# Autodesk Inventor assembly: carriage
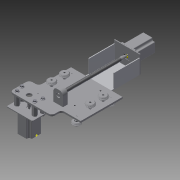
[picture p0: Inventor's stored thumbnail of the model, 180x180]
Saved by Autodesk Inventor 2013 (Build 170138000, 138)
## iProperties
Created: 2012-12-03
Part Number: carriage
Document SubType Name: Weldment
Designer: Istvan
Weld Material: Aluminum 6061, Welded
Mass: 772.809 g
Surface Area: 2087.48 cm^2
Volume: 764.052 cm^3
Density: 1.01146 g/cm^3
Author: Istvan
## Documents named in this file (14)
- C:\Users\james.eddlestone\Documents\GitHub\Crown-Fire\CAD\Carriage\carriage.iam
- C:\Users\james.eddlestone\Documents\GitHub\Crown-Fire\CAD\Carriage\backplate.ipt
- C:\Users\james.eddlestone\Documents\GitHub\Crown-Fire\CAD\Hardware\Bearings\DualVee-size2.ipt
- C:\Users\james.eddlestone\Documents\GitHub\Crown-Fire\CAD\Electronics\Motors\G723-280-4.ipt
- C:\Users\james.eddlestone\Documents\GitHub\Crown-Fire\CAD\Carriage\zMotorMount.ipt
- C:\Users\james.eddlestone\Documents\GitHub\Crown-Fire\CAD\Carriage\acmeScrew.ipt
- C:\Users\james.eddlestone\Documents\GitHub\Crown-Fire\CAD\Hardware\motorCoupling.ipt
- C:\Users\james.eddlestone\Documents\GitHub\Crown-Fire\CAD\Carriage\acmeBearingBlock.ipt
- C:\Users\james.eddlestone\Documents\GitHub\Crown-Fire\CAD\Carriage\motorMount.ipt
- C:\Users\james.eddlestone\Documents\GitHub\Crown-Fire\CAD\Hardware\1-4-20Standoff.ipt
- C:\Users\james.eddlestone\Documents\GitHub\Crown-Fire\CAD\Hardware\Fasteners\IFI 111 - 1_4-20 UNC x 0.5.ipt
- C:\Users\james.eddlestone\Documents\GitHub\Crown-Fire\CAD\Hardware\Bearings\10mm-double.ipt
- C:\Users\james.eddlestone\Documents\GitHub\Crown-Fire\CAD\CuttingHead\motorTower.ipt
- C:\Users\istvan.burbank\Documents\GitHub\Crown-Fire\CAD\Templates\channel2.25x4.ipt
## Components (31 placed, 12 different names)
1. backplate:1 — Mate:18, Mate:19, Mate:20, Mate:21, Mate:22, Mate:23, Mate:24, Mate:25, Mate:32, Mate:33, Mate:34, Mate:35, Mate:36, Insert:35, Mate:46, Insert:36, Insert:37, Insert:38, Insert:39, Mate:49, Flush:7, Mate:50, Flush:10
2. DualVee-size2:1 — Mate:18
3. DualVee-size2:2 — Mate:19
4. DualVee-size2:3 — Mate:21
5. DualVee-size2:4 — Mate:20
6. G723-280-4:1 — Mate:6, Mate:7, Mate:8, Mate:10, Flush:6, Angle:3
7. zMotorMount:1 — Mate:6, Mate:7, Angle:3, Mate:51, Flush:8, Flush:9
8. acmeScrew:1 — Mate:9, Mate:10, Flush:6, Mate:12, Mate:40, Mate:41, Mate:44
9. motorCoupling:1 — Mate:8, Mate:9, Mate:44
10. acmeBearingBlock:1 — Mate:12, Mate:39, Mate:49, Flush:7
11. DualVee-size2:5 — Mate:24
12. DualVee-size2:6 — Mate:23
13. DualVee-size2:7 — Mate:25
14. DualVee-size2:8 — Mate:22
15. G723-280-4:2 — Mate:31, Mate:32, Insert:32, Mate:45, Angle:2
16. motorMount:1 — Insert:19, Insert:20, Insert:28, Insert:29, Insert:30, Insert:31, Mate:45, Insert:33, Insert:34, Angle:2
17. motorCoupling:2 — Mate:31, Insert:32
18. 1-4-20Standoff:1 — Mate:35, Insert:34
19. 1-4-20Standoff:2 — Mate:33, Insert:33
20. 1-4-20Standoff:3 — Mate:36, Insert:29, Mate:46
21. 1-4-20Standoff:4 — Mate:34, Insert:28, Insert:35
22. Hex Flange Screw - Inch (IFI) 1/4-20 UNC x 0.5:1 — Insert:20
23. Hex Flange Screw - Inch (IFI) 1/4-20 UNC x 0.5:2 — Insert:19
24. Hex Flange Screw - Inch (IFI) 1/4-20 UNC x 0.5:3 — Insert:30
25. Hex Flange Screw - Inch (IFI) 1/4-20 UNC x 0.5:4 — Insert:31
26. Hex Flange Screw - Inch (IFI) 1/4-20 UNC x 0.5:5 — Insert:39
27. Hex Flange Screw - Inch (IFI) 1/4-20 UNC x 0.5:6 — Insert:37
28. Hex Flange Screw - Inch (IFI) 1/4-20 UNC x 0.5:7 — Insert:38
29. Hex Flange Screw - Inch (IFI) 1/4-20 UNC x 0.5:8 — Insert:36
30. 10mm-double:1 — Mate:39, Mate:40, Mate:41
31. motorTower:1 — Mate:50, Mate:51, Flush:8, Flush:9, Flush:10
## Relationships (50: Mate 29, Insert 14, Flush 5, Angle 2)
- Mate:6: G723-280-4:1 ↔ zMotorMount:1
- Mate:7: G723-280-4:1 ↔ zMotorMount:1
- Mate:8: G723-280-4:1 ↔ motorCoupling:1
- Mate:9: acmeScrew:1 ↔ motorCoupling:1
- Mate:10: G723-280-4:1 ↔ acmeScrew:1
- Flush:6: G723-280-4:1 ↔ acmeScrew:1
- Mate:12: acmeScrew:1 ↔ acmeBearingBlock:1
- Mate:18: backplate:1 ↔ DualVee-size2:1
- Mate:19: backplate:1 ↔ DualVee-size2:2
- Mate:20: backplate:1 ↔ DualVee-size2:4
- Mate:21: backplate:1 ↔ DualVee-size2:3
- Mate:22: backplate:1 ↔ DualVee-size2:8
- Mate:23: backplate:1 ↔ DualVee-size2:6
- Mate:24: backplate:1 ↔ DualVee-size2:5
- Mate:25: backplate:1 ↔ DualVee-size2:7
- Mate:31: G723-280-4:2 ↔ motorCoupling:2
- Mate:32: backplate:1 ↔ G723-280-4:2
- Mate:33: backplate:1 ↔ 1-4-20Standoff:2
- Mate:34: backplate:1 ↔ 1-4-20Standoff:4
- Mate:35: backplate:1 ↔ 1-4-20Standoff:1
- Mate:36: backplate:1 ↔ 1-4-20Standoff:3
- Insert:19: motorMount:1 ↔ Hex Flange Screw - Inch (IFI) 1/4-20 UNC x 0.5:2
- Insert:20: motorMount:1 ↔ Hex Flange Screw - Inch (IFI) 1/4-20 UNC x 0.5:1
- Insert:28: motorMount:1 ↔ 1-4-20Standoff:4
- Insert:29: motorMount:1 ↔ 1-4-20Standoff:3
- Insert:30: motorMount:1 ↔ Hex Flange Screw - Inch (IFI) 1/4-20 UNC x 0.5:3
- Insert:31: motorMount:1 ↔ Hex Flange Screw - Inch (IFI) 1/4-20 UNC x 0.5:4
- Insert:32 (-12.7 mm): G723-280-4:2 ↔ motorCoupling:2
- Mate:39: acmeBearingBlock:1 ↔ 10mm-double:1
- Mate:40: acmeScrew:1 ↔ 10mm-double:1
- Mate:41: acmeScrew:1 ↔ 10mm-double:1
- Mate:44: acmeScrew:1 ↔ motorCoupling:1
- Mate:45: G723-280-4:2 ↔ motorMount:1
- Insert:33: motorMount:1 ↔ 1-4-20Standoff:2
- Insert:34: motorMount:1 ↔ 1-4-20Standoff:1
- Insert:35: backplate:1 ↔ 1-4-20Standoff:4
- Mate:46: backplate:1 ↔ 1-4-20Standoff:3
- Insert:36: backplate:1 ↔ Hex Flange Screw - Inch (IFI) 1/4-20 UNC x 0.5:8
- Insert:37: backplate:1 ↔ Hex Flange Screw - Inch (IFI) 1/4-20 UNC x 0.5:6
- Insert:38: backplate:1 ↔ Hex Flange Screw - Inch (IFI) 1/4-20 UNC x 0.5:7
- Insert:39: backplate:1 ↔ Hex Flange Screw - Inch (IFI) 1/4-20 UNC x 0.5:5
- Angle:2 (0 deg): G723-280-4:2 ↔ motorMount:1
- Mate:49: backplate:1 ↔ acmeBearingBlock:1
- Angle:3 (0 deg): G723-280-4:1 ↔ zMotorMount:1
- Flush:7 (50.8 mm): backplate:1 ↔ acmeBearingBlock:1
- Mate:50: backplate:1 ↔ motorTower:1
- Mate:51: zMotorMount:1 ↔ motorTower:1
- Flush:8: zMotorMount:1 ↔ motorTower:1
- Flush:9: zMotorMount:1 ↔ motorTower:1
- Flush:10 (50.8 mm): backplate:1 ↔ motorTower:1
